# Autodesk Inventor assembly: FrontWheelAssembly
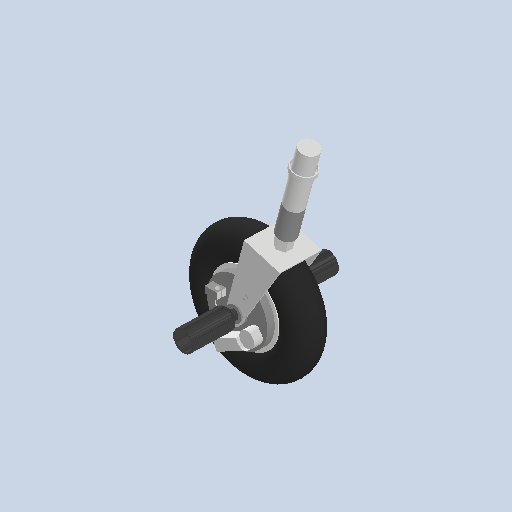
[picture p0: Inventor's stored thumbnail of the model, 512x512]
Saved by Autodesk Inventor 2022.2 (Build 262287010, 287A)
## iProperties
Created: 2022-04-08
Part Number: FrontWheelAssembly
Document SubType Name: Assembly
Designer: Finn Oriwohl
Author: Finn Oriwohl
## Documents named in this file (5)
- C:\Users\Finn Oriwohl\Documents\htx\1g g\BeerCart-CAD-Inventor\Workspaces\Workspace\FrontWheelAssembly.iam
- C:\Users\Finn Oriwohl\Documents\htx\1g g\BeerCart-CAD-Inventor\Workspaces\Workspace\frontwheelFork.ipt
- C:\Users\Finn Oriwohl\Documents\htx\1g g\BeerCart-CAD-Inventor\Workspaces\Workspace\FreeBackWheel.ipt
- C:\Users\Finn Oriwohl\Documents\htx\1g g\BeerCart-CAD-Inventor\Workspaces\Workspace\pegsFront wheel.ipt
- C:\Users\Finn Oriwohl\Documents\htx\1g g\BeerCart-CAD-Inventor\Workspaces\Workspace\headset bearing.ipt
## Components (5 placed, 4 different names)
1. headset bearing:1
2. frontwheelFork:1
3. FreeBackWheel:1
4. pegsFront wheel:1
5. pegsFront wheel:2
## Relationships (3: Insert 3)
- [Insert] (-5 mm): frontwheelFork:1 ↔ FreeBackWheel:1
- [Insert]: frontwheelFork:1 ↔ pegsFront wheel:1
- [Insert]: frontwheelFork:1 ↔ pegsFront wheel:2
